# Autodesk Inventor assembly: roller bushing
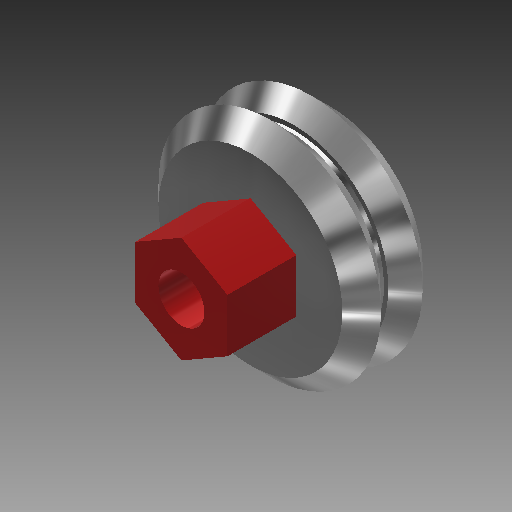
[picture p0: Inventor's stored thumbnail of the model, 512x512]
Saved by Autodesk Inventor 2017 SP1 (Build 210196100, 196)
## iProperties
Created: 2018-01-19
Part Number: roller bushing
Document SubType Name: Assembly
Designer: Ben
Mass: 50.3375 g
Surface Area: 39.965 cm^2
Volume: 7.45623 cm^3
Density: 6.75107 g/cm^3
Author: Ben
## Documents named in this file (3)
- C:\Users\Ben\Desktop\Projects\2018 Robot\Cube Lift\roller bushing.iam
- C:\Users\Ben\Desktop\Projects\2018 Robot\Cube Lift\roller.ipt
- C:\Users\Ben\Desktop\Projects\2018 Robot\Cube Lift\bushing.ipt
## Components (2 placed, 2 different names)
1. roller:1 — Flush:1, Flush:2, Flush:3, Insert:1
2. bushing:1 — Insert:1
## Relationships (4: Flush 3, Insert 1)
- Flush:1: roller:1
- Flush:2: roller:1
- Flush:3: roller:1
- Insert:1: roller:1 ↔ bushing:1
